# Autodesk Inventor assembly: Head_camera_frame
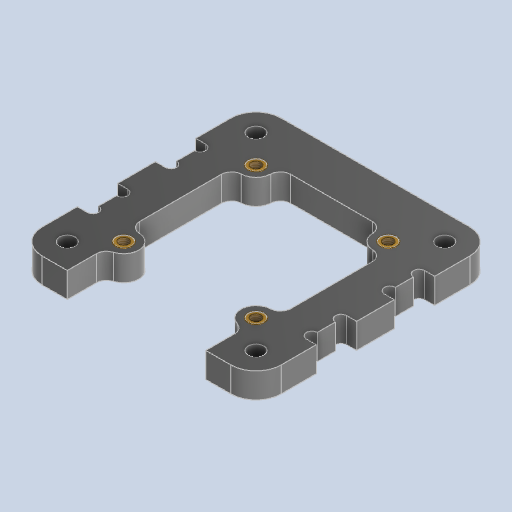
[picture p0: Inventor's stored thumbnail of the model, 512x512]
Saved by Autodesk Inventor 2022.3 (Build 263350000, 350)
## iProperties
Created: 2023-04-07
Part Number: Head_camera_frame
Document SubType Name: Assembly
Designer: Masato Kubotera
Author: Masato Kubotera
## Documents named in this file (3)
- C:\Users\Masato\Documents\Inventor\Inventor for CIT Brains\SUSTAINA-OP - mod\UpperBody\Head\Head_camera_frame.iam
- C:\Users\Masato\Documents\Inventor\Inventor for CIT Brains\SUSTAINA-OP - mod\UpperBody\Head\Head_camera_frame.ipt
- C:\Users\Masato\Documents\Inventor\Inventor for CIT Brains\SUSTAINA-OP - mod\ReadyMade\InsertNut\BRM2-4.1.ipt
## Components (5 placed, 2 different names)
1. Head_camera_frame:1 — フラッシュ:1, フラッシュ:2, フラッシュ:3, 挿入:1, 挿入:2, 挿入:3, 挿入:4
2. BRM2-4.1:1 — 挿入:1
3. BRM2-4.1:2 — 挿入:2
4. BRM2-4.1:3 — 挿入:3
5. BRM2-4.1:4 — 挿入:4
## Relationships (7: Insert 4, Flush 3)
- フラッシュ:1 [Flush]: Head_camera_frame:1
- フラッシュ:2 [Flush]: Head_camera_frame:1
- フラッシュ:3 [Flush]: Head_camera_frame:1
- 挿入:1 [Insert]: Head_camera_frame:1 ↔ BRM2-4.1:1
- 挿入:2 [Insert]: Head_camera_frame:1 ↔ BRM2-4.1:2
- 挿入:3 [Insert]: Head_camera_frame:1 ↔ BRM2-4.1:3
- 挿入:4 [Insert]: Head_camera_frame:1 ↔ BRM2-4.1:4
